# Autodesk Inventor assembly: ShieldAssembly
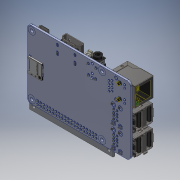
[picture p0: Inventor's stored thumbnail of the model, 180x180]
Saved by Autodesk Inventor 2017 (Build 210142000, 142)
## iProperties
Created: 2017-06-22
Part Number: ShieldAssembly
Document SubType Name: Assembly
Designer: P. Baesso
Author: P. Baesso
## Documents named in this file (3)
- C:\Rymapt\ethoscope_hardware\core_Rymapt\Shield\ShieldAssembly.iam
- C:\Rymapt\ethoscope_hardware\core\RPi3\RPi3_ModelB.ipt
- C:\Rymapt\ethoscope_hardware\core_Rymapt\Shield\ShieldBare.ipt
## Components (2 placed, 2 different names)
1. RPi3_ModelB:1 — Flush:1
2. ShieldBare:1 — Flush:1
## Relationships (1: Flush 1)
- Flush:1: RPi3_ModelB:1 ↔ ShieldBare:1
